# Autodesk Inventor assembly: 200-60-DIFFERENTIAL-CONNECTOR-02
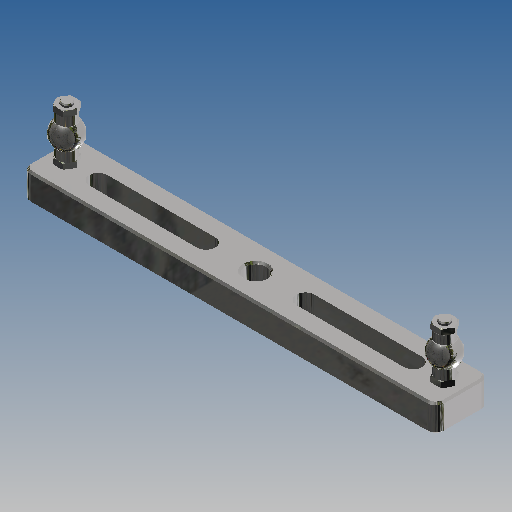
[picture p0: Inventor's stored thumbnail of the model, 512x512]
Saved by Autodesk Inventor 2018.2 (Build 222227000, 227)
## iProperties
Manager: feesmrt
Company: FRANC0R
Created: 2017-12-19
Part Number: 200-60-DIFFERENTIAL-CONNECTOR-02
Project: Rescue Robot
Cost Center: -
Material: Generisch
Document SubType Name: Assembly
Designer: feesmrt
Engineer: feesmrt
Authority: feesmrt
Description: Differential Connector Arm
Stock Number: 200-60-DIFFERENTIAL-CONNECTOR-02
Subject: Rescue Robot
Author: feesmrt
Revision Number: 1
Title: Differential Connector Arm
## Documents named in this file (6)
- C:\Users\feesmrt\Documents\FRANC0R\CAD\02-Rocker-Bogie-Robot\200-ROCKER-BOGIE\200-60-DIFFERENTIAL\200-60-DIFFERENTIAL-CONNECTOR-02.iam
- C:\Users\feesmrt\Documents\FRANC0R\CAD\02-Rocker-Bogie-Robot\200-ROCKER-BOGIE\200-60-DIFFERENTIAL\200-60-DIFFERENTIAL-CONNECTOR-01.ipt
- C:\Users\feesmrt\Documents\FRANC0R\CAD\02-Rocker-Bogie-Robot\200-ROCKER-BOGIE\200-60-DIFFERENTIAL\200-60-DIFFERENTIAL-BAR-02.ipt
- C:\Users\feesmrt\Documents\FRANC0R\CAD\02-Rocker-Bogie-Robot\900-COMPONENTS\900-41-NUTS\900-41-NUTS-ISO4035-M6.ipt
- C:\Users\feesmrt\Documents\FRANC0R\CAD\02-Rocker-Bogie-Robot\900-COMPONENTS\900-70-ANGLE-JOINTS\900-70-ANGLE-JOINT-DIN648-M8-2.ipt
- C:\Users\feesmrt\Documents\FRANC0R\CAD\02-Rocker-Bogie-Robot\200-ROCKER-BOGIE\200-60-DIFFERENTIAL\200-60-DIFFERENTIAL-BAR-04.ipt
## Components (11 placed, 5 different names)
1. 200-60-DIFFERENTIAL-CONNECTOR-01:1 — Passend:1, Passend:2, Passend:5, Passend:6
2. 200-60-DIFFERENTIAL-BAR-02:1 — Passend:2, Passend:3, Passend:7, Passend:9, Passend:12, Passend:13, Passend:17
3. 200-60-DIFFERENTIAL-BAR-02:2 — Passend:1, Passend:4, Passend:8, Passend:10, Passend:11, Passend:14, Passend:19
4. 900-41-NUTS-ISO4035-M6:1 — Passend:3, Passend:6, Passend:7
5. 900-41-NUTS-ISO4035-M6:2 — Passend:4, Passend:5, Passend:8
6. 900-70-ANGLE-JOINT-DIN648-M8-2:1 — Passend:9, Passend:12, Passend:16
7. 900-70-ANGLE-JOINT-DIN648-M8-2:2 — Passend:10, Passend:11, Passend:15
8. 200-60-DIFFERENTIAL-BAR-04:1 — Passend:13, Passend:16, Passend:18
9. 200-60-DIFFERENTIAL-BAR-04:2 — Passend:14, Passend:15, Passend:20
10. 900-41-NUTS-ISO4035-M6:3 — Passend:17, Passend:18
11. 900-41-NUTS-ISO4035-M6:4 — Passend:19, Passend:20
## Relationships (20: Mate 20)
- Passend:1 [Mate]: 200-60-DIFFERENTIAL-CONNECTOR-01:1 ↔ 200-60-DIFFERENTIAL-BAR-02:2
- Passend:2 [Mate]: 200-60-DIFFERENTIAL-CONNECTOR-01:1 ↔ 200-60-DIFFERENTIAL-BAR-02:1
- Passend:3 [Mate]: 200-60-DIFFERENTIAL-BAR-02:1 ↔ 900-41-NUTS-ISO4035-M6:1
- Passend:4 [Mate]: 200-60-DIFFERENTIAL-BAR-02:2 ↔ 900-41-NUTS-ISO4035-M6:2
- Passend:5 [Mate]: 200-60-DIFFERENTIAL-CONNECTOR-01:1 ↔ 900-41-NUTS-ISO4035-M6:2
- Passend:6 [Mate]: 200-60-DIFFERENTIAL-CONNECTOR-01:1 ↔ 900-41-NUTS-ISO4035-M6:1
- Passend:7 [Mate]: 200-60-DIFFERENTIAL-BAR-02:1 ↔ 900-41-NUTS-ISO4035-M6:1
- Passend:8 [Mate]: 200-60-DIFFERENTIAL-BAR-02:2 ↔ 900-41-NUTS-ISO4035-M6:2
- Passend:9 [Mate]: 200-60-DIFFERENTIAL-BAR-02:1 ↔ 900-70-ANGLE-JOINT-DIN648-M8-2:1
- Passend:10 [Mate]: 200-60-DIFFERENTIAL-BAR-02:2 ↔ 900-70-ANGLE-JOINT-DIN648-M8-2:2
- Passend:11 [Mate]: 200-60-DIFFERENTIAL-BAR-02:2 ↔ 900-70-ANGLE-JOINT-DIN648-M8-2:2
- Passend:12 [Mate]: 200-60-DIFFERENTIAL-BAR-02:1 ↔ 900-70-ANGLE-JOINT-DIN648-M8-2:1
- Passend:13 [Mate]: 200-60-DIFFERENTIAL-BAR-02:1 ↔ 200-60-DIFFERENTIAL-BAR-04:1
- Passend:14 [Mate]: 200-60-DIFFERENTIAL-BAR-02:2 ↔ 200-60-DIFFERENTIAL-BAR-04:2
- Passend:15 [Mate]: 900-70-ANGLE-JOINT-DIN648-M8-2:2 ↔ 200-60-DIFFERENTIAL-BAR-04:2
- Passend:16 [Mate]: 900-70-ANGLE-JOINT-DIN648-M8-2:1 ↔ 200-60-DIFFERENTIAL-BAR-04:1
- Passend:17 [Mate]: 200-60-DIFFERENTIAL-BAR-02:1 ↔ 900-41-NUTS-ISO4035-M6:3
- Passend:18 [Mate]: 200-60-DIFFERENTIAL-BAR-04:1 ↔ 900-41-NUTS-ISO4035-M6:3
- Passend:19 [Mate]: 200-60-DIFFERENTIAL-BAR-02:2 ↔ 900-41-NUTS-ISO4035-M6:4
- Passend:20 [Mate]: 200-60-DIFFERENTIAL-BAR-04:2 ↔ 900-41-NUTS-ISO4035-M6:4
